# Autodesk Inventor assembly: joint_meteor
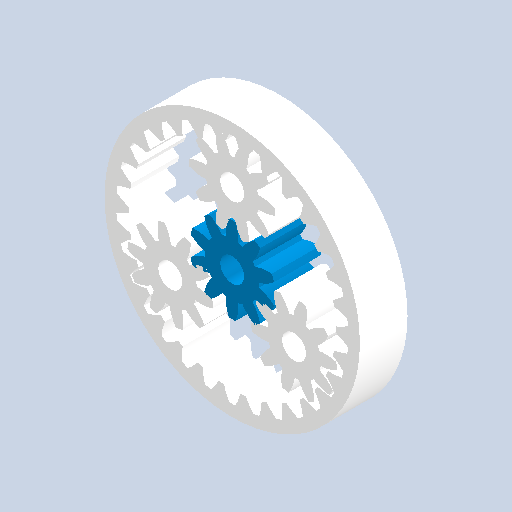
[picture p0: Inventor's stored thumbnail of the model, 512x512]
Saved by Autodesk Inventor 2025.3 (Build 293356030, 356C)
## iProperties
Created: 2025-09-07
Part Number: joint_meteor
Document SubType Name: Assembly
Designer: MSI
Mass: 145.812 g
Surface Area: 544.297 cm^2
Volume: 118.547 cm^3
Density: 1.23 g/cm^3
Author: MSI
## Documents named in this file (5)
- C:\Users\MSI\Desktop\Project\11. 로봇팔\Robot Arm Model\Robot_Arm_6_v1\joint3_meteor.iam
- C:\Users\MSI\Desktop\Project\11. 로봇팔\Robot Arm Model\Robot_Arm_6_v1\joint3_sun.ipt
- C:\Users\MSI\Desktop\Project\11. 로봇팔\Robot Arm Model\Robot_Arm_6_v1\joint3_planet.ipt
- C:\Users\MSI\Desktop\Project\11. 로봇팔\Robot Arm Model\Robot_Arm_6_v1\joint3_ring.ipt
- C:\Users\MSI\Desktop\Project\11. 로봇팔\Robot Arm Model\Robot_Arm_6_v1\joint3_carrier.ipt
## Components (6 placed, 3 different names)
1. 스퍼 기어2:1 — 강체:1, 강체:5
2. 스퍼 기어1:1 — 강체:2
3. 스퍼 기어2:2 — 강체:5
4. 스퍼 기어1:2 — 강체:4
5. 스퍼 기어1:3 — 강체:3
6. joint3_carrier:1 — 강체:1, 강체:2, 강체:3, 강체:4
## Relationships (5: WeldJoint 5)
- 강체:1 [WeldJoint]: 스퍼 기어2:1 ↔ joint3_carrier:1
- 강체:2 [WeldJoint]: 스퍼 기어1:1 ↔ joint3_carrier:1
- 강체:3 [WeldJoint]: 스퍼 기어1:3 ↔ joint3_carrier:1
- 강체:4 [WeldJoint]: 스퍼 기어1:2 ↔ joint3_carrier:1
- 강체:5 [WeldJoint]: 스퍼 기어2:1 ↔ 스퍼 기어2:2
